# Autodesk Inventor assembly: MH5Lmontagem oficial
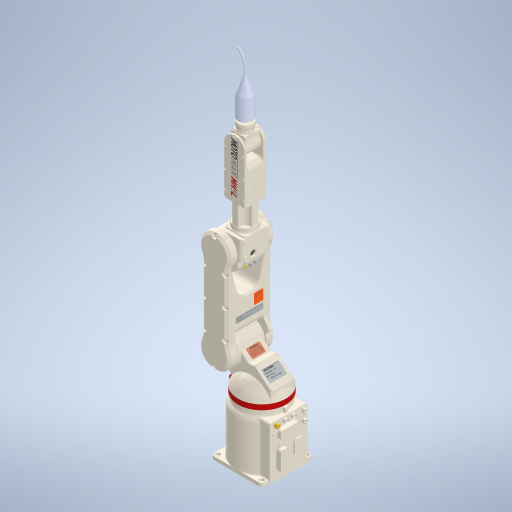
[picture p0: Inventor's stored thumbnail of the model, 512x512]
Saved by Autodesk Inventor 2023 (Build 270158000, 158)
## iProperties
Created: 2012-10-02
Part Number: MH5Lmontagem oficial
Document SubType Name: Assembly
Designer: kleber
Sending System: SolidWorks 2012
Last Author: Márcio Amorim
Last Saved: 2012-10-03
Author: kleber
## Documents named in this file (8)
- C:\Users\klebe\OneDrive\Documents\GitHub\Sala-braquiterapia\Sala de Braquiterapia\Inventor\MH5Lmontagem oficial.iam
- C:\Users\klebe\OneDrive\Documents\GitHub\Sala-braquiterapia\Sala de Braquiterapia\Inventor\MH5Lbase do robo.iam
- C:\Users\klebe\OneDrive\Documents\GitHub\Sala-braquiterapia\Sala de Braquiterapia\Inventor\MH5Lbraço 1.iam
- C:\Users\klebe\OneDrive\Documents\GitHub\Sala-braquiterapia\Sala de Braquiterapia\Inventor\MH5Lbraço 2.iam
- C:\Users\klebe\OneDrive\Documents\GitHub\Sala-braquiterapia\Sala de Braquiterapia\Inventor\MH5Lbraço 3.iam
- C:\Users\klebe\OneDrive\Documents\GitHub\Sala-braquiterapia\Sala de Braquiterapia\Inventor\MH5Lbraço 4.ipt
- C:\Users\klebe\OneDrive\Documents\GitHub\Sala-braquiterapia\Sala de Braquiterapia\Inventor\MH5Lbraço 5.ipt
- C:\Users\klebe\OneDrive\Documents\GitHub\Sala-braquiterapia\Sala de Braquiterapia\Inventor\Mateus]\Ferramenta de succao\succaoFerramenta2.0 agr vai.ipt
## Components (7 placed, 7 different names)
1. base do robo:1 [sub-assembly] — Rotational:1, Mate:1, Mate:2, Angle:3
2. braço 1:1 [sub-assembly] — Rotational:1, Rotational:2
3. braço 2:1 [sub-assembly] — Rotational:2, Rotational:3, Angle:1, Angle:2, Angle:3
4. braço 3:1 [sub-assembly] — Rotational:3, Rotational:4
5. MH5Lbraço 4:1 — Rotational:4, Rotational:5, Angle:1, Angle:2, Angle:4
6. MH5Lbraço 5:1 — Rotational:5, Angle:4, Rotational:6
7. succaoFerramenta2.0 agr vai:1 — Rotational:6
## Relationships (12: RevoluteJoint 6, Angle 4, Mate 2)
- Rotational:1 [RevoluteJoint]: base do robo:1 ↔ braço 1:1
- Rotational:2 [RevoluteJoint]: braço 1:1 ↔ braço 2:1
- Rotational:3 [RevoluteJoint] (7 mm): braço 2:1 ↔ braço 3:1
- Rotational:4 [RevoluteJoint]: braço 3:1 ↔ MH5Lbraço 4:1
- Rotational:5 [RevoluteJoint]: MH5Lbraço 4:1 ↔ MH5Lbraço 5:1
- Mate:1: base do robo:1
- Mate:2: base do robo:1
- Angle:1 (180 deg): braço 2:1 ↔ MH5Lbraço 4:1
- Angle:2 (0 deg): braço 2:1 ↔ MH5Lbraço 4:1
- Angle:3 (0 deg): base do robo:1 ↔ braço 2:1
- Angle:4 (0 deg): MH5Lbraço 4:1 ↔ MH5Lbraço 5:1
- Rotational:6 [RevoluteJoint]: MH5Lbraço 5:1 ↔ succaoFerramenta2.0 agr vai:1
